# Autodesk Inventor assembly: BV-ASM-222-100 copy
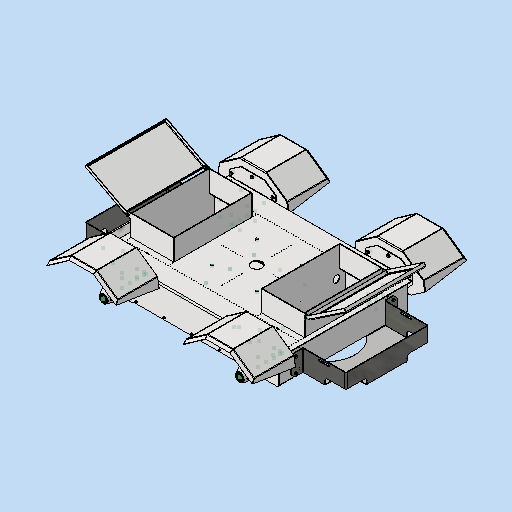
[picture p0: Inventor's stored thumbnail of the model, 512x512]
Saved by Autodesk Inventor 2025.3 (Build 293356030, 356C)
## iProperties
Created: 2025-12-05
Part Number: BV-ASM-222-100 copy
Document SubType Name: Assembly
Designer: josh
Mass: 150717 g
Surface Area: 81479.7 cm^2
Volume: 19199.6 cm^3
Density: 7.85 g/cm^3
Description: BASE VEHICLE COMPLETE ASSEMBLY
Author: josh
## iProperties of the stored document MemberDocs/x54frrunuJ0si20qmEdadrqylTg
Created: 2025-12-05
Part Number: BV-ASM-222-100 wip
Document SubType Name: Assembly
Designer: josh
Mass: 150717 g
Surface Area: 81479.7 cm^2
Volume: 19199.6 cm^3
Density: 7.85 g/cm^3
Description: BASE VEHICLE COMPLETE ASSEMBLY
Author: josh
## iProperties of the stored document MemberDocs/xFojfi5agHc25u2sk4sonpsnbLc
Created: 2025-12-05
Part Number: BV-ASM-222-100 wip
Document SubType Name: Assembly
Designer: josh
Mass: 150717 g
Surface Area: 81479.7 cm^2
Volume: 19199.6 cm^3
Density: 7.85 g/cm^3
Description: BASE VEHICLE COMPLETE ASSEMBLY
Author: josh
## Documents named in this file (59)
- R:\A1- Neuweg Design Data\OM Robotics\BASE VEHICLE DESIGN PROJECT\BV-ASM-222-100 copy.iam
- R:\A1- Neuweg Design Data\OM Robotics\BASE VEHICLE DESIGN PROJECT\BV-222-105.ipt
- R:\A1- Neuweg Design Data\OM Robotics\BASE VEHICLE DESIGN PROJECT\BV-222-106.ipt
- R:\A1- Neuweg Design Data\OM Robotics\BASE VEHICLE DESIGN PROJECT\BV-222-107.ipt
- R:\A1- Neuweg Design Data\OM Robotics\BASE VEHICLE DESIGN PROJECT\BV-222-108.ipt
- R:\A1- Neuweg Design Data\OM Robotics\BASE VEHICLE DESIGN PROJECT\BV-222-109.ipt
- R:\A1- Neuweg Design Data\OM Robotics\BASE VEHICLE DESIGN PROJECT\BV-222-112.ipt
- R:\A1- Neuweg Design Data\OM Robotics\BASE VEHICLE DESIGN PROJECT\BV-222-116.ipt
- R:\A1- Neuweg Design Data\OM Robotics\BASE VEHICLE DESIGN PROJECT\BV-222-117.ipt
- R:\A1- Neuweg Design Data\OM Robotics\BASE VEHICLE DESIGN PROJECT\BV-222-118.ipt
- R:\A1- Neuweg Design Data\OM Robotics\BASE VEHICLE DESIGN PROJECT\BV-222-119.ipt
- R:\A1- Neuweg Design Data\OM Robotics\BASE VEHICLE DESIGN PROJECT\BV-222-120.ipt
- R:\A1- Neuweg Design Data\OM Robotics\BASE VEHICLE DESIGN PROJECT\0222-110.ipt
- R:\A1- Neuweg Design Data\OM Robotics\BASE VEHICLE DESIGN PROJECT\3_8-16 x 5_8 Flange Bolt.ipt
- R:\A1- Neuweg Design Data\OM Robotics\BASE VEHICLE DESIGN PROJECT\1_4-20 UNC x 0.625.ipt
- R:\A1- Neuweg Design Data\OM Robotics\BASE VEHICLE DESIGN PROJECT\90128A277.ipt
- R:\A1- Neuweg Design Data\OM Robotics\BASE VEHICLE DESIGN PROJECT\91290A446.ipt
- R:\A1- Neuweg Design Data\OM Robotics\BASE VEHICLE DESIGN PROJECT\91259A177.ipt
- R:\A1- Neuweg Design Data\OM Robotics\BASE VEHICLE DESIGN PROJECT\94945A213.ipt
- R:\A1- Neuweg Design Data\OM Robotics\BASE VEHICLE DESIGN PROJECT\BV-ASM-222-102.iam
- R:\A1- Neuweg Design Data\OM Robotics\BASE VEHICLE DESIGN PROJECT\30205.ipt
- R:\A1- Neuweg Design Data\OM Robotics\BASE VEHICLE DESIGN PROJECT\251105 Motor_Drive.ipt
- R:\A1- Neuweg Design Data\OM Robotics\BASE VEHICLE DESIGN PROJECT\22x10x8.ipt
- R:\A1- Neuweg Design Data\OM Robotics\BASE VEHICLE DESIGN PROJECT\0222-113-2.ipt
- R:\A1- Neuweg Design Data\OM Robotics\BASE VEHICLE DESIGN PROJECT\97260A109.ipt
- R:\A1- Neuweg Design Data\OM Robotics\BASE VEHICLE DESIGN PROJECT\93560A112.ipt
- R:\A1- Neuweg Design Data\OM Robotics\BASE VEHICLE DESIGN PROJECT\1199N323.ipt
- R:\A1- Neuweg Design Data\OM Robotics\BASE VEHICLE DESIGN PROJECT\BV-ASM-222-103.iam
- R:\A1- Neuweg Design Data\OM Robotics\BASE VEHICLE DESIGN PROJECT\BV-ASM-222-104.iam
- R:\A1- Neuweg Design Data\OM Robotics\BASE VEHICLE DESIGN PROJECT\BV-ASM-222-105.iam
- C:\WORK\INVENTOR PROJECTS\misc custom projects\O&M ROBOTICS\ROBOT BASE VEHICLE\BV-222-105.ipt
- C:\WORK\INVENTOR PROJECTS\misc custom projects\O&M ROBOTICS\ROBOT BASE VEHICLE\BV-222-106.ipt
- C:\WORK\INVENTOR PROJECTS\misc custom projects\O&M ROBOTICS\ROBOT BASE VEHICLE\BV-222-107.ipt
- C:\WORK\INVENTOR PROJECTS\misc custom projects\O&M ROBOTICS\ROBOT BASE VEHICLE\BV-222-108.ipt
- C:\WORK\INVENTOR PROJECTS\misc custom projects\O&M ROBOTICS\ROBOT BASE VEHICLE\BV-222-109.ipt
- C:\WORK\INVENTOR PROJECTS\misc custom projects\O&M ROBOTICS\ROBOT BASE VEHICLE\BV-222-112.ipt
- C:\WORK\INVENTOR PROJECTS\misc custom projects\O&M ROBOTICS\ROBOT BASE VEHICLE\BV-222-116.ipt
- C:\WORK\INVENTOR PROJECTS\misc custom projects\O&M ROBOTICS\ROBOT BASE VEHICLE\BV-222-117.ipt
- C:\WORK\INVENTOR PROJECTS\misc custom projects\O&M ROBOTICS\ROBOT BASE VEHICLE\BV-222-118.ipt
- C:\WORK\INVENTOR PROJECTS\misc custom projects\O&M ROBOTICS\ROBOT BASE VEHICLE\BV-222-119.ipt
- C:\WORK\INVENTOR PROJECTS\misc custom projects\O&M ROBOTICS\ROBOT BASE VEHICLE\BV-222-120.ipt
- C:\WORK\INVENTOR PROJECTS\misc custom projects\O&M ROBOTICS\ROBOT BASE VEHICLE\0222-110.ipt
- C:\WORK\INVENTOR PROJECTS\misc custom projects\O&M ROBOTICS\ROBOT BASE VEHICLE\3_8-16 x 5_8 Flange Bolt.ipt
- C:\WORK\INVENTOR PROJECTS\misc custom projects\O&M ROBOTICS\ROBOT BASE VEHICLE\1_4-20 UNC x 0.625.ipt
- C:\WORK\INVENTOR PROJECTS\misc custom projects\O&M ROBOTICS\ROBOT BASE VEHICLE\90128A277\90128A277\90128A277.ipt
- C:\WORK\INVENTOR PROJECTS\misc custom projects\O&M ROBOTICS\ROBOT BASE VEHICLE\91290A446\91290A446\91290A446.ipt
- C:\WORK\INVENTOR PROJECTS\misc custom projects\O&M ROBOTICS\ROBOT BASE VEHICLE\91259A177\91259A177\91259A177.ipt
- C:\WORK\INVENTOR PROJECTS\misc custom projects\O&M ROBOTICS\ROBOT BASE VEHICLE\94945A213\94945A213\94945A213.ipt
- C:\WORK\INVENTOR PROJECTS\misc custom projects\O&M ROBOTICS\ROBOT BASE VEHICLE\BV-ASM-222-102.iam
- C:\WORK\INVENTOR PROJECTS\misc custom projects\O&M ROBOTICS\ROBOT BASE VEHICLE\30205\30205\30205.ipt
- C:\WORK\INVENTOR PROJECTS\misc custom projects\O&M ROBOTICS\ROBOT BASE VEHICLE\251105 Motor_Drive.ipt
- C:\WORK\INVENTOR PROJECTS\misc custom projects\O&M ROBOTICS\ROBOT BASE VEHICLE\22x10x8.ipt
- C:\WORK\INVENTOR PROJECTS\misc custom projects\O&M ROBOTICS\ROBOT BASE VEHICLE\0222-113-2.ipt
- C:\WORK\INVENTOR PROJECTS\misc custom projects\O&M ROBOTICS\ROBOT BASE VEHICLE\97260A109.ipt
- C:\WORK\INVENTOR PROJECTS\misc custom projects\O&M ROBOTICS\ROBOT BASE VEHICLE\93560A112_Steel Hex Weld Nut\93560A112_Steel Hex Weld Nut\93560A112.ipt
- C:\WORK\INVENTOR PROJECTS\misc custom projects\O&M ROBOTICS\ROBOT BASE VEHICLE\1199N323\1199N323\1199N323.ipt
- C:\WORK\INVENTOR PROJECTS\misc custom projects\O&M ROBOTICS\ROBOT BASE VEHICLE\BV-ASM-222-103.iam
- C:\WORK\INVENTOR PROJECTS\misc custom projects\O&M ROBOTICS\ROBOT BASE VEHICLE\BV-ASM-222-104.iam
- C:\WORK\INVENTOR PROJECTS\misc custom projects\O&M ROBOTICS\ROBOT BASE VEHICLE\BV-ASM-222-105.iam
## Components (199 placed, 29 different names)
1. BV-ASM-222-104:1 [sub-assembly] — Flush:11, Flush:12, Flush:13
2. BV-ASM-222-105:1 [sub-assembly] — Mate:105
3. BV-ASM-222-103:1 [sub-assembly] — Flush:8, Flush:9, Flush:10, Insert:201, Insert:202
4. BV-ASM-222-103:2 [sub-assembly] — Insert:203, Insert:204, Insert:205, Insert:206, Insert:219, Insert:220
5. BV-ASM-222-103:3 [sub-assembly] — Insert:207, Insert:208, Insert:209, Insert:210, Insert:221, Insert:222
6. BV-ASM-222-103:4 [sub-assembly] — Insert:211, Insert:212, Insert:213, Insert:214, Insert:223, Insert:224
7. BV-222-105:1 — Insert:117, Insert:118, Insert:119, Insert:120, Insert:121, Insert:122, Insert:123, Insert:124, Insert:125, Insert:126, Insert:127, Insert:128
8. BV-222-106:1 — Mate:2, Insert:162, Insert:166
9. BV-222-107:1 — Insert:161, Insert:165
10. BV-222-108:1 — Mate:2, Flush:1, Mate:3
11. BV-222-109:1 — Insert:75, Insert:76, Insert:77, Insert:201, Insert:202
12. BV-222-112:1 — Mate:73, Mate:74, Mate:75, Mate:76, Mate:77, Mate:78, Mate:79, Mate:80, Mate:81, Mate:82, Mate:83, Mate:84, Mate:85, Mate:86, Mate:87, Mate:88, Mate:89, Mate:90, Mate:91, Mate:92
13. BV-222-116:1 — Insert:174, Insert:189
14. BV-222-118:1
15. BV-222-119:1 — Insert:175, Insert:190
16. BV-222-120:1 — Mate:5
17. BV-222-112:3
18. BV-222-106:2 — Mate:1, Insert:163, Insert:168
19. BV-222-107:2 — Insert:164, Insert:167
20. BV-222-108:2 — Mate:1, Mate:3
21. BV-222-109:2 — Insert:78, Insert:79, Insert:80, Insert:203, Insert:204, Insert:219, Insert:220
22. BV-222-116:2 — Insert:173, Insert:185
23. BV-222-118:2
24. BV-222-119:2 — Insert:176, Insert:186
25. BV-222-120:2
26. BV-222-109:3 — Insert:81, Insert:82, Insert:83, Insert:211, Insert:212, Insert:223, Insert:224
27. BV-222-116:3 — Insert:170, Insert:192
28. BV-222-118:3
29. BV-222-119:3 — Insert:169, Insert:191
30. BV-222-120:3 — Mate:14
31. BV-222-109:4 — Insert:84, Insert:85, Insert:86, Insert:207, Insert:208, Insert:221, Insert:222
32. BV-222-116:4 — Insert:172, Insert:188
33. BV-222-118:4
34. BV-222-119:4 — Insert:171, Insert:187
35. BV-222-120:4 — Mate:11
36. BV-ASM-222-102:1 [sub-assembly] — Mate:12, Mate:13, Insert:30, Insert:31, Insert:215
37. BV-ASM-222-102:2 [sub-assembly] — Mate:4, Mate:6, Insert:16, Insert:17, Mate:102, Insert:217
38. BV-ASM-222-102:3 [sub-assembly] — Mate:9, Mate:10, Insert:28, Insert:29, Mate:103, Insert:218
39. BV-ASM-222-102:4 [sub-assembly] — Mate:7, Mate:8, Insert:22, Insert:23, Mate:101, Insert:216
40. 251105 Motor_Drive:1 — Mate:4, Mate:5, Mate:6, Flush:2, Flush:3, Mate:102
41. 22x10x8:1 — Insert:16, Insert:17
42. 97260A109:1 — Insert:196
43. 251105 Motor_Drive:2 — Mate:7, Flush:2, Flush:3, Mate:8, Flush:4, Mate:101
44. 97260A109:2 — Insert:194
45. 22x10x8:2 — Insert:22, Insert:23
46. 251105 Motor_Drive:3 — Mate:9, Mate:10, Mate:11, Flush:4, Flush:5, Mate:103
47. 251105 Motor_Drive:4 — Mate:12, Mate:13, Mate:14, Flush:5
48. 97260A109:3 — Insert:200
49. 97260A109:4 — Insert:198
50. 22x10x8:3 — Insert:28, Insert:29
51. 22x10x8:4 — Insert:30, Insert:31
52. 93560A112:1
53. 93560A112:2
54. 93560A112:3
55. 93560A112:4
56. 0222-110:1 — Mate:104, Flush:7
57. 0222-110:2 — Flush:7, Flush:19, Mate:105
58. Hex Flange Screw - Inch (IFI) 3/8-16 UNC x 0.625:9
59. Hex Flange Screw - Inch (IFI) 3/8-16 UNC x 0.625:10
60. Hex Flange Screw - Inch (IFI) 3/8-16 UNC x 0.625:11
61. Hex Flange Screw - Inch (IFI) 3/8-16 UNC x 0.625:12
62. Hex Flange Screw - Inch (IFI) 3/8-16 UNC x 0.625:13
63. Hex Flange Screw - Inch (IFI) 3/8-16 UNC x 0.625:14
64. Hex Flange Screw - Inch (IFI) 3/8-16 UNC x 0.625:15
65. Hex Flange Screw - Inch (IFI) 3/8-16 UNC x 0.625:16
66. Hex Flange Screw - Inch (IFI) 3/8-16 UNC x 0.625:18 — Insert:75, Mate:21, Mate:22
67. Hex Flange Screw - Inch (IFI) 3/8-16 UNC x 0.625:19 — Insert:76, Mate:21, Mate:22
68. Hex Flange Screw - Inch (IFI) 3/8-16 UNC x 0.625:20 — Insert:77, Mate:23, Mate:24
69. Hex Flange Screw - Inch (IFI) 3/8-16 UNC x 0.625:21 — Insert:78, Mate:23, Mate:24
70. Hex Flange Screw - Inch (IFI) 3/8-16 UNC x 0.625:22 — Insert:79, Mate:25, Mate:26
71. Hex Flange Screw - Inch (IFI) 3/8-16 UNC x 0.625:23 — Insert:80, Mate:25, Mate:26
72. Hex Flange Screw - Inch (IFI) 3/8-16 UNC x 0.625:24 — Insert:81, Mate:27, Mate:28
73. Hex Flange Screw - Inch (IFI) 3/8-16 UNC x 0.625:25 — Insert:82, Mate:27, Mate:28
74. Hex Flange Screw - Inch (IFI) 3/8-16 UNC x 0.625:26 — Insert:83, Mate:29, Mate:30
75. Hex Flange Screw - Inch (IFI) 3/8-16 UNC x 0.625:27 — Insert:84, Mate:29, Mate:30
76. Hex Flange Screw - Inch (IFI) 3/8-16 UNC x 0.625:28 — Insert:85, Mate:31, Mate:32
77. Hex Flange Screw - Inch (IFI) 3/8-16 UNC x 0.625:29 — Insert:86, Mate:31, Mate:32
78. Hex Flange Screw - Inch (IFI) 3/8-16 UNC x 0.625:30 — Mate:33, Mate:34
79. Hex Flange Screw - Inch (IFI) 3/8-16 UNC x 0.625:31 — Mate:33, Mate:34
80. Hex Flange Screw - Inch (IFI) 3/8-16 UNC x 0.625:32 — Mate:35, Mate:36, Insert:205
81. Hex Flange Screw - Inch (IFI) 3/8-16 UNC x 0.625:33 — Mate:35, Mate:36, Insert:206
82. Hex Flange Screw - Inch (IFI) 3/8-16 UNC x 0.625:34 — Mate:37, Mate:38, Insert:214
83. Hex Flange Screw - Inch (IFI) 3/8-16 UNC x 0.625:35 — Mate:37, Mate:38, Insert:213
84. Hex Flange Screw - Inch (IFI) 3/8-16 UNC x 0.625:36 — Mate:39, Mate:40, Insert:209
85. Hex Flange Screw - Inch (IFI) 3/8-16 UNC x 0.625:37 — Mate:39, Mate:40, Insert:210
86. 1_4-20 UNC x 0.625:1 — Mate:41, Mate:42
87. 1_4-20 UNC x 0.625:2 — Mate:41, Mate:42
88. 1_4-20 UNC x 0.625:3 — Mate:43, Mate:44
89. 1_4-20 UNC x 0.625:4 — Mate:43, Mate:44
90. 1_4-20 UNC x 0.625:5 — Mate:45, Mate:46
91. 1_4-20 UNC x 0.625:6 — Mate:45, Mate:46
92. 1_4-20 UNC x 0.625:7 — Mate:47, Mate:48
93. 1_4-20 UNC x 0.625:8 — Mate:47, Mate:48
94. 1_4-20 UNC x 0.625:9 — Mate:49, Mate:50
95. 1_4-20 UNC x 0.625:10 — Mate:49, Mate:50
96. Hex Flange Screw - Inch (IFI) 3/8-16 UNC x 0.625:38 — Insert:117, Mate:51, Mate:52
97. Hex Flange Screw - Inch (IFI) 3/8-16 UNC x 0.625:39 — Insert:118, Mate:51, Mate:52
98. Hex Flange Screw - Inch (IFI) 3/8-16 UNC x 0.625:40 — Insert:119, Mate:53, Mate:54
99. Hex Flange Screw - Inch (IFI) 3/8-16 UNC x 0.625:41 — Insert:120, Mate:53, Mate:54
100. Hex Flange Screw - Inch (IFI) 3/8-16 UNC x 0.625:42 — Insert:121, Mate:55, Mate:56
101. Hex Flange Screw - Inch (IFI) 3/8-16 UNC x 0.625:43 — Insert:122, Mate:55, Mate:56
102. Hex Flange Screw - Inch (IFI) 3/8-16 UNC x 0.625:44 — Insert:123, Mate:57, Mate:58
103. Hex Flange Screw - Inch (IFI) 3/8-16 UNC x 0.625:45 — Insert:124, Mate:57, Mate:58
104. Hex Flange Screw - Inch (IFI) 3/8-16 UNC x 0.625:46 — Insert:125, Mate:59, Mate:60
105. Hex Flange Screw - Inch (IFI) 3/8-16 UNC x 0.625:47 — Insert:126, Mate:59, Mate:60
106. Hex Flange Screw - Inch (IFI) 3/8-16 UNC x 0.625:48 — Insert:127, Mate:61, Mate:62
107. Hex Flange Screw - Inch (IFI) 3/8-16 UNC x 0.625:49 — Insert:128, Mate:61, Mate:62
108. 1_4-20 UNC x 0.625:11 — Mate:75, Mate:76
109. 1_4-20 UNC x 0.625:12 — Mate:89, Mate:90
110. 1_4-20 UNC x 0.625:13 — Mate:77, Mate:78
111. 1_4-20 UNC x 0.625:14 — Mate:81, Mate:82
112. 1_4-20 UNC x 0.625:15 — Mate:79, Mate:80
113. 1_4-20 UNC x 0.625:16 — Mate:91, Mate:92
114. 1_4-20 UNC x 0.625:17 — Mate:85, Mate:86
115. 1_4-20 UNC x 0.625:18 — Mate:83, Mate:84
116. 1_4-20 UNC x 0.625:19 — Mate:87, Mate:88
117. 1_4-20 UNC x 0.625:20 — Mate:73, Mate:74
118. 1_4-20 UNC x 0.625:21 — Mate:93, Mate:94
119. 1_4-20 UNC x 0.625:22 — Mate:93, Mate:94
120. 1_4-20 UNC x 0.625:23 — Mate:95, Mate:96
121. 1_4-20 UNC x 0.625:24 — Mate:95, Mate:96
122. 1_4-20 UNC x 0.625:25
123. 1_4-20 UNC x 0.625:26
124. 1_4-20 UNC x 0.625:27 — Mate:97, Mate:98
125. 1_4-20 UNC x 0.625:28 — Mate:97, Mate:98
126. 1_4-20 UNC x 0.625:29 — Mate:99, Mate:100
127. 1_4-20 UNC x 0.625:30 — Mate:99, Mate:100
128. 90128A277:1
129. 90128A277:2
130. 90128A277:3
131. 90128A277:4
132. 90128A277:5
133. 90128A277:6
134. 90128A277:7
135. 90128A277:8
136. 90128A277:9
137. 90128A277:10
138. 90128A277:11
139. 90128A277:12
140. 90128A277:13
141. 90128A277:14
142. 90128A277:15
143. 90128A277:16
144. 91290A446:1
145. 91290A446:2
146. 91290A446:3
147. 91290A446:4
148. 91290A446:5
149. 91290A446:6
150. 91290A446:7
151. 91290A446:8
152. 91290A446:9
153. 91290A446:10
154. 91290A446:11
155. 91290A446:12
156. 91290A446:13
157. 91290A446:14
158. 91290A446:15
159. 91290A446:16
160. 91259A177:1 — Insert:162
161. 91259A177:2 — Insert:161
162. 91259A177:3 — Insert:163
163. 91259A177:4 — Insert:164
164. 94945A213:1 — Insert:165
165. 94945A213:2 — Insert:166
166. 94945A213:3 — Insert:167
167. 94945A213:4 — Insert:168
168. 30205:1 — Insert:170, Insert:215
169. 30205:2 — Insert:169, Insert:197
170. 30205:3 — Insert:172, Insert:218
171. 30205:4 — Insert:171, Insert:199
172. 30205:5 — Insert:176, Insert:193
173. 30205:6 — Insert:173, Insert:216
174. 30205:7 — Insert:175, Insert:195
175. 30205:8 — Insert:174, Insert:217
176. 0222-113-2:1 — Insert:199, Insert:200
177. 0222-113-2:2 — Insert:193, Insert:194
178. 0222-113-2:3 — Insert:197, Insert:198
179. 0222-113-2:4 — Insert:195, Insert:196
180. 1199N323:1 — Insert:185
181. 1199N323:2 — Insert:186
182. 1199N323:3 — Insert:187
183. 1199N323:4 — Insert:188
184. 1199N323:5 — Insert:189
185. 1199N323:6 — Insert:190
186. 1199N323:7 — Insert:191
187. 1199N323:8 — Insert:192
188. BV-222-117:1
189. BV-222-117:2
190. BV-222-117:3
191. BV-222-117:4
192. BV-222-117:5
193. BV-222-117:6
194. BV-222-117:7
195. BV-222-117:9
196. BV-222-117:10
197. BV-222-117:8
198. BV-222-117:11
199. BV-222-117:12
## Component patterns: (3 elements, first: BV-222-117:1), (3 elements, first: BV-222-117:4), (3 elements, first: BV-222-117:7), (3 elements, first: BV-222-117:8)
## Relationships (259: Insert 146, Mate 99, Flush 13, Angle 1)
- [Insert]: BV-ASM-222-104:1 ↔ BV-222-112:3
- [Insert]: BV-ASM-222-104:1 ↔ BV-222-112:3
- Mate:1: BV-222-106:2 ↔ BV-222-108:2
- Mate:2: BV-222-106:1 ↔ BV-222-108:1
- Flush:1: BV-222-108:1
- Mate:3: BV-222-108:1 ↔ BV-222-108:2
- Mate:4: BV-ASM-222-102:2 ↔ 251105 Motor_Drive:1
- Mate:5: BV-222-120:1 ↔ 251105 Motor_Drive:1
- Mate:6: BV-ASM-222-102:2 ↔ 251105 Motor_Drive:1
- Insert:16: BV-ASM-222-102:2 ↔ 22x10x8:1
- Insert:17: BV-ASM-222-102:2 ↔ 22x10x8:1
- [Angle] (-90 deg): BV-ASM-222-105:1 ↔ 251105 Motor_Drive:1
- Mate:7: BV-ASM-222-102:4 ↔ 251105 Motor_Drive:2
- Flush:2: 251105 Motor_Drive:1 ↔ 251105 Motor_Drive:2
- Flush:3: 251105 Motor_Drive:1 ↔ 251105 Motor_Drive:2
- Mate:8: BV-ASM-222-102:4 ↔ 251105 Motor_Drive:2
- Insert:22: BV-ASM-222-102:4 ↔ 22x10x8:2
- Insert:23: BV-ASM-222-102:4 ↔ 22x10x8:2
- Mate:9: BV-ASM-222-102:3 ↔ 251105 Motor_Drive:3
- Mate:10: BV-ASM-222-102:3 ↔ 251105 Motor_Drive:3
- Mate:11: BV-222-120:4 ↔ 251105 Motor_Drive:3
- Flush:4: 251105 Motor_Drive:2 ↔ 251105 Motor_Drive:3
- Mate:12: BV-ASM-222-102:1 ↔ 251105 Motor_Drive:4
- Mate:13: BV-ASM-222-102:1 ↔ 251105 Motor_Drive:4
- Mate:14: BV-222-120:3 ↔ 251105 Motor_Drive:4
- Flush:5: 251105 Motor_Drive:3 ↔ 251105 Motor_Drive:4
- Insert:28: BV-ASM-222-102:3 ↔ 22x10x8:3
- Insert:29: BV-ASM-222-102:3 ↔ 22x10x8:3
- Insert:30: BV-ASM-222-102:1 ↔ 22x10x8:4
- Insert:31: BV-ASM-222-102:1 ↔ 22x10x8:4
- [Insert]: BV-ASM-222-105:1 ↔ 93560A112:1
- [Insert]: BV-ASM-222-105:1 ↔ 93560A112:2
- [Insert]: BV-ASM-222-105:1 ↔ 93560A112:3
- [Insert]: BV-ASM-222-105:1 ↔ 93560A112:4
- [Mate]: BV-ASM-222-105:1 ↔ 0222-110:1
- Mate:104: 0222-110:1
- [Mate]: BV-ASM-222-105:1 ↔ 0222-110:1
- Flush:7: 0222-110:1 ↔ 0222-110:2
- Flush:19: 0222-110:2
- [Insert] (4.7752 mm): BV-ASM-222-105:1 ↔ Hex Flange Screw - Inch (IFI) 3/8-16 UNC x 0.625:9
- [Insert] (4.7752 mm): BV-ASM-222-105:1 ↔ Hex Flange Screw - Inch (IFI) 3/8-16 UNC x 0.625:10
- [Insert] (4.7752 mm): BV-ASM-222-105:1 ↔ Hex Flange Screw - Inch (IFI) 3/8-16 UNC x 0.625:12
- [Insert] (4.7752 mm): BV-ASM-222-105:1 ↔ Hex Flange Screw - Inch (IFI) 3/8-16 UNC x 0.625:11
- [Insert] (4.7752 mm): BV-ASM-222-105:1 ↔ Hex Flange Screw - Inch (IFI) 3/8-16 UNC x 0.625:16
- [Insert] (4.7752 mm): BV-ASM-222-105:1 ↔ Hex Flange Screw - Inch (IFI) 3/8-16 UNC x 0.625:15
- [Insert] (4.7752 mm): BV-ASM-222-105:1 ↔ Hex Flange Screw - Inch (IFI) 3/8-16 UNC x 0.625:14
- [Insert] (4.7752 mm): BV-ASM-222-105:1 ↔ Hex Flange Screw - Inch (IFI) 3/8-16 UNC x 0.625:13
- Insert:75: BV-222-109:1 ↔ Hex Flange Screw - Inch (IFI) 3/8-16 UNC x 0.625:18
- Insert:76: BV-222-109:1 ↔ Hex Flange Screw - Inch (IFI) 3/8-16 UNC x 0.625:19
- Mate:21: Hex Flange Screw - Inch (IFI) 3/8-16 UNC x 0.625:18 ↔ Hex Flange Screw - Inch (IFI) 3/8-16 UNC x 0.625:19
- Mate:22: Hex Flange Screw - Inch (IFI) 3/8-16 UNC x 0.625:18 ↔ Hex Flange Screw - Inch (IFI) 3/8-16 UNC x 0.625:19
- Insert:77: BV-222-109:1 ↔ Hex Flange Screw - Inch (IFI) 3/8-16 UNC x 0.625:20
- Insert:78: BV-222-109:2 ↔ Hex Flange Screw - Inch (IFI) 3/8-16 UNC x 0.625:21
- Mate:23: Hex Flange Screw - Inch (IFI) 3/8-16 UNC x 0.625:20 ↔ Hex Flange Screw - Inch (IFI) 3/8-16 UNC x 0.625:21
- Mate:24: Hex Flange Screw - Inch (IFI) 3/8-16 UNC x 0.625:20 ↔ Hex Flange Screw - Inch (IFI) 3/8-16 UNC x 0.625:21
- Insert:79: BV-222-109:2 ↔ Hex Flange Screw - Inch (IFI) 3/8-16 UNC x 0.625:22
- Insert:80: BV-222-109:2 ↔ Hex Flange Screw - Inch (IFI) 3/8-16 UNC x 0.625:23
- Mate:25: Hex Flange Screw - Inch (IFI) 3/8-16 UNC x 0.625:22 ↔ Hex Flange Screw - Inch (IFI) 3/8-16 UNC x 0.625:23
- Mate:26: Hex Flange Screw - Inch (IFI) 3/8-16 UNC x 0.625:22 ↔ Hex Flange Screw - Inch (IFI) 3/8-16 UNC x 0.625:23
- Insert:81: BV-222-109:3 ↔ Hex Flange Screw - Inch (IFI) 3/8-16 UNC x 0.625:24
- Insert:82: BV-222-109:3 ↔ Hex Flange Screw - Inch (IFI) 3/8-16 UNC x 0.625:25
- Mate:27: Hex Flange Screw - Inch (IFI) 3/8-16 UNC x 0.625:24 ↔ Hex Flange Screw - Inch (IFI) 3/8-16 UNC x 0.625:25
- Mate:28: Hex Flange Screw - Inch (IFI) 3/8-16 UNC x 0.625:24 ↔ Hex Flange Screw - Inch (IFI) 3/8-16 UNC x 0.625:25
- Insert:83: BV-222-109:3 ↔ Hex Flange Screw - Inch (IFI) 3/8-16 UNC x 0.625:26
- Insert:84: BV-222-109:4 ↔ Hex Flange Screw - Inch (IFI) 3/8-16 UNC x 0.625:27
- Mate:29: Hex Flange Screw - Inch (IFI) 3/8-16 UNC x 0.625:26 ↔ Hex Flange Screw - Inch (IFI) 3/8-16 UNC x 0.625:27
- Mate:30: Hex Flange Screw - Inch (IFI) 3/8-16 UNC x 0.625:26 ↔ Hex Flange Screw - Inch (IFI) 3/8-16 UNC x 0.625:27
- Insert:85: BV-222-109:4 ↔ Hex Flange Screw - Inch (IFI) 3/8-16 UNC x 0.625:28
- Insert:86: BV-222-109:4 ↔ Hex Flange Screw - Inch (IFI) 3/8-16 UNC x 0.625:29
- Mate:31: Hex Flange Screw - Inch (IFI) 3/8-16 UNC x 0.625:28 ↔ Hex Flange Screw - Inch (IFI) 3/8-16 UNC x 0.625:29
- Mate:32: Hex Flange Screw - Inch (IFI) 3/8-16 UNC x 0.625:28 ↔ Hex Flange Screw - Inch (IFI) 3/8-16 UNC x 0.625:29
- [Insert]: BV-ASM-222-103:1 ↔ Hex Flange Screw - Inch (IFI) 3/8-16 UNC x 0.625:30
- [Insert]: BV-ASM-222-103:1 ↔ Hex Flange Screw - Inch (IFI) 3/8-16 UNC x 0.625:31
- Mate:33: Hex Flange Screw - Inch (IFI) 3/8-16 UNC x 0.625:30 ↔ Hex Flange Screw - Inch (IFI) 3/8-16 UNC x 0.625:31
- Mate:34: Hex Flange Screw - Inch (IFI) 3/8-16 UNC x 0.625:30 ↔ Hex Flange Screw - Inch (IFI) 3/8-16 UNC x 0.625:31
- Mate:35: Hex Flange Screw - Inch (IFI) 3/8-16 UNC x 0.625:32 ↔ Hex Flange Screw - Inch (IFI) 3/8-16 UNC x 0.625:33
- Mate:36: Hex Flange Screw - Inch (IFI) 3/8-16 UNC x 0.625:32 ↔ Hex Flange Screw - Inch (IFI) 3/8-16 UNC x 0.625:33
- Mate:37: Hex Flange Screw - Inch (IFI) 3/8-16 UNC x 0.625:34 ↔ Hex Flange Screw - Inch (IFI) 3/8-16 UNC x 0.625:35
- Mate:38: Hex Flange Screw - Inch (IFI) 3/8-16 UNC x 0.625:34 ↔ Hex Flange Screw - Inch (IFI) 3/8-16 UNC x 0.625:35
- Mate:39: Hex Flange Screw - Inch (IFI) 3/8-16 UNC x 0.625:36 ↔ Hex Flange Screw - Inch (IFI) 3/8-16 UNC x 0.625:37
- Mate:40: Hex Flange Screw - Inch (IFI) 3/8-16 UNC x 0.625:36 ↔ Hex Flange Screw - Inch (IFI) 3/8-16 UNC x 0.625:37
- [Insert]: BV-ASM-222-104:1 ↔ 1_4-20 UNC x 0.625:1
- [Insert]: BV-ASM-222-104:1 ↔ 1_4-20 UNC x 0.625:2
- Mate:41: 1_4-20 UNC x 0.625:1 ↔ 1_4-20 UNC x 0.625:2
- Mate:42: 1_4-20 UNC x 0.625:1 ↔ 1_4-20 UNC x 0.625:2
- [Insert]: BV-ASM-222-104:1 ↔ 1_4-20 UNC x 0.625:3
- [Insert]: BV-ASM-222-104:1 ↔ 1_4-20 UNC x 0.625:4
- Mate:43: 1_4-20 UNC x 0.625:3 ↔ 1_4-20 UNC x 0.625:4
- Mate:44: 1_4-20 UNC x 0.625:3 ↔ 1_4-20 UNC x 0.625:4
- [Insert]: BV-ASM-222-104:1 ↔ 1_4-20 UNC x 0.625:5
- [Insert]: BV-ASM-222-104:1 ↔ 1_4-20 UNC x 0.625:6
- Mate:45: 1_4-20 UNC x 0.625:5 ↔ 1_4-20 UNC x 0.625:6
- Mate:46: 1_4-20 UNC x 0.625:5 ↔ 1_4-20 UNC x 0.625:6
- [Insert]: BV-ASM-222-104:1 ↔ 1_4-20 UNC x 0.625:7
- [Insert]: BV-ASM-222-104:1 ↔ 1_4-20 UNC x 0.625:8
- Mate:47: 1_4-20 UNC x 0.625:7 ↔ 1_4-20 UNC x 0.625:8
- Mate:48: 1_4-20 UNC x 0.625:7 ↔ 1_4-20 UNC x 0.625:8
- [Insert]: BV-ASM-222-104:1 ↔ 1_4-20 UNC x 0.625:9
- [Insert]: BV-ASM-222-104:1 ↔ 1_4-20 UNC x 0.625:10
- Mate:49: 1_4-20 UNC x 0.625:9 ↔ 1_4-20 UNC x 0.625:10
- Mate:50: 1_4-20 UNC x 0.625:9 ↔ 1_4-20 UNC x 0.625:10
- Insert:117: BV-222-105:1 ↔ Hex Flange Screw - Inch (IFI) 3/8-16 UNC x 0.625:38
- Insert:118: BV-222-105:1 ↔ Hex Flange Screw - Inch (IFI) 3/8-16 UNC x 0.625:39
- Mate:51: Hex Flange Screw - Inch (IFI) 3/8-16 UNC x 0.625:38 ↔ Hex Flange Screw - Inch (IFI) 3/8-16 UNC x 0.625:39
- Mate:52: Hex Flange Screw - Inch (IFI) 3/8-16 UNC x 0.625:38 ↔ Hex Flange Screw - Inch (IFI) 3/8-16 UNC x 0.625:39
- Insert:119: BV-222-105:1 ↔ Hex Flange Screw - Inch (IFI) 3/8-16 UNC x 0.625:40
- Insert:120: BV-222-105:1 ↔ Hex Flange Screw - Inch (IFI) 3/8-16 UNC x 0.625:41
- Mate:53: Hex Flange Screw - Inch (IFI) 3/8-16 UNC x 0.625:40 ↔ Hex Flange Screw - Inch (IFI) 3/8-16 UNC x 0.625:41
- Mate:54: Hex Flange Screw - Inch (IFI) 3/8-16 UNC x 0.625:40 ↔ Hex Flange Screw - Inch (IFI) 3/8-16 UNC x 0.625:41
- Insert:121: BV-222-105:1 ↔ Hex Flange Screw - Inch (IFI) 3/8-16 UNC x 0.625:42
- Insert:122: BV-222-105:1 ↔ Hex Flange Screw - Inch (IFI) 3/8-16 UNC x 0.625:43
- Mate:55: Hex Flange Screw - Inch (IFI) 3/8-16 UNC x 0.625:42 ↔ Hex Flange Screw - Inch (IFI) 3/8-16 UNC x 0.625:43
- Mate:56: Hex Flange Screw - Inch (IFI) 3/8-16 UNC x 0.625:42 ↔ Hex Flange Screw - Inch (IFI) 3/8-16 UNC x 0.625:43
- Insert:123: BV-222-105:1 ↔ Hex Flange Screw - Inch (IFI) 3/8-16 UNC x 0.625:44
- Insert:124: BV-222-105:1 ↔ Hex Flange Screw - Inch (IFI) 3/8-16 UNC x 0.625:45
- Mate:57: Hex Flange Screw - Inch (IFI) 3/8-16 UNC x 0.625:44 ↔ Hex Flange Screw - Inch (IFI) 3/8-16 UNC x 0.625:45
- Mate:58: Hex Flange Screw - Inch (IFI) 3/8-16 UNC x 0.625:44 ↔ Hex Flange Screw - Inch (IFI) 3/8-16 UNC x 0.625:45
- Insert:125: BV-222-105:1 ↔ Hex Flange Screw - Inch (IFI) 3/8-16 UNC x 0.625:46
- Insert:126: BV-222-105:1 ↔ Hex Flange Screw - Inch (IFI) 3/8-16 UNC x 0.625:47
- Mate:59: Hex Flange Screw - Inch (IFI) 3/8-16 UNC x 0.625:46 ↔ Hex Flange Screw - Inch (IFI) 3/8-16 UNC x 0.625:47
- Mate:60: Hex Flange Screw - Inch (IFI) 3/8-16 UNC x 0.625:46 ↔ Hex Flange Screw - Inch (IFI) 3/8-16 UNC x 0.625:47
- Insert:127: BV-222-105:1 ↔ Hex Flange Screw - Inch (IFI) 3/8-16 UNC x 0.625:48
- Insert:128: BV-222-105:1 ↔ Hex Flange Screw - Inch (IFI) 3/8-16 UNC x 0.625:49
- Mate:61: Hex Flange Screw - Inch (IFI) 3/8-16 UNC x 0.625:48 ↔ Hex Flange Screw - Inch (IFI) 3/8-16 UNC x 0.625:49
- Mate:62: Hex Flange Screw - Inch (IFI) 3/8-16 UNC x 0.625:48 ↔ Hex Flange Screw - Inch (IFI) 3/8-16 UNC x 0.625:49
- [Mate]: 1_4-20 UNC x 0.625:11 ↔ 1_4-20 UNC x 0.625:12
- [Mate]: 1_4-20 UNC x 0.625:11 ↔ 1_4-20 UNC x 0.625:12
- [Mate]: 1_4-20 UNC x 0.625:13 ↔ 1_4-20 UNC x 0.625:14
- [Mate]: 1_4-20 UNC x 0.625:13 ↔ 1_4-20 UNC x 0.625:14
- [Mate]: 1_4-20 UNC x 0.625:17 ↔ 1_4-20 UNC x 0.625:18
- [Mate]: 1_4-20 UNC x 0.625:17 ↔ 1_4-20 UNC x 0.625:18
- [Mate]: 1_4-20 UNC x 0.625:19 ↔ 1_4-20 UNC x 0.625:20
- [Mate]: 1_4-20 UNC x 0.625:19 ↔ 1_4-20 UNC x 0.625:20
- Mate:73: BV-222-112:1 ↔ 1_4-20 UNC x 0.625:20
- Mate:74: BV-222-112:1 ↔ 1_4-20 UNC x 0.625:20
- Mate:75: BV-222-112:1 ↔ 1_4-20 UNC x 0.625:11
- Mate:76: BV-222-112:1 ↔ 1_4-20 UNC x 0.625:11
- Mate:77: BV-222-112:1 ↔ 1_4-20 UNC x 0.625:13
- Mate:78: BV-222-112:1 ↔ 1_4-20 UNC x 0.625:13
- Mate:79: BV-222-112:1 ↔ 1_4-20 UNC x 0.625:15
- Mate:80: BV-222-112:1 ↔ 1_4-20 UNC x 0.625:15
- Mate:81: BV-222-112:1 ↔ 1_4-20 UNC x 0.625:14
- Mate:82: BV-222-112:1 ↔ 1_4-20 UNC x 0.625:14
- Mate:83: BV-222-112:1 ↔ 1_4-20 UNC x 0.625:18
- Mate:84: BV-222-112:1 ↔ 1_4-20 UNC x 0.625:18
- Mate:85: BV-222-112:1 ↔ 1_4-20 UNC x 0.625:17
- Mate:86: BV-222-112:1 ↔ 1_4-20 UNC x 0.625:17
- Mate:87: BV-222-112:1 ↔ 1_4-20 UNC x 0.625:19
- Mate:88: BV-222-112:1 ↔ 1_4-20 UNC x 0.625:19
- Mate:89: BV-222-112:1 ↔ 1_4-20 UNC x 0.625:12
- Mate:90: BV-222-112:1 ↔ 1_4-20 UNC x 0.625:12
- Mate:91: BV-222-112:1 ↔ 1_4-20 UNC x 0.625:16
- Mate:92: BV-222-112:1 ↔ 1_4-20 UNC x 0.625:16
- Mate:93: 1_4-20 UNC x 0.625:21 ↔ 1_4-20 UNC x 0.625:22
- Mate:94: 1_4-20 UNC x 0.625:21 ↔ 1_4-20 UNC x 0.625:22
- Mate:95: 1_4-20 UNC x 0.625:23 ↔ 1_4-20 UNC x 0.625:24
- Mate:96: 1_4-20 UNC x 0.625:23 ↔ 1_4-20 UNC x 0.625:24
- Mate:97: 1_4-20 UNC x 0.625:27 ↔ 1_4-20 UNC x 0.625:28
- Mate:98: 1_4-20 UNC x 0.625:27 ↔ 1_4-20 UNC x 0.625:28
- Mate:99: 1_4-20 UNC x 0.625:29 ↔ 1_4-20 UNC x 0.625:30
- Mate:100: 1_4-20 UNC x 0.625:29 ↔ 1_4-20 UNC x 0.625:30
- [Insert]: BV-ASM-222-104:1 ↔ 90128A277:1
- [Insert]: BV-ASM-222-104:1 ↔ 90128A277:2
- [Insert]: BV-ASM-222-104:1 ↔ 90128A277:3
- [Insert]: BV-ASM-222-104:1 ↔ 90128A277:4
- [Insert]: BV-ASM-222-104:1 ↔ 90128A277:5
- [Insert]: BV-ASM-222-104:1 ↔ 90128A277:6
- [Insert]: BV-ASM-222-104:1 ↔ 90128A277:7
- [Insert]: BV-ASM-222-104:1 ↔ 90128A277:8
- [Insert]: BV-ASM-222-104:1 ↔ 90128A277:9
- [Insert]: BV-ASM-222-104:1 ↔ 90128A277:10
- [Insert]: BV-ASM-222-104:1 ↔ 90128A277:11
- [Insert]: BV-ASM-222-104:1 ↔ 90128A277:12
- [Insert]: BV-ASM-222-104:1 ↔ 90128A277:13
- [Insert]: BV-ASM-222-104:1 ↔ 90128A277:14
- [Insert]: BV-ASM-222-104:1 ↔ 90128A277:15
- [Insert]: BV-ASM-222-104:1 ↔ 90128A277:16
- [Insert]: BV-ASM-222-105:1 ↔ 91290A446:1
- [Insert]: BV-ASM-222-105:1 ↔ 91290A446:2
- [Insert]: BV-ASM-222-105:1 ↔ 91290A446:3
- [Insert]: BV-ASM-222-105:1 ↔ 91290A446:4
- [Insert]: BV-ASM-222-105:1 ↔ 91290A446:5
- [Insert]: BV-ASM-222-105:1 ↔ 91290A446:6
- [Insert]: BV-ASM-222-105:1 ↔ 91290A446:7
- [Insert]: BV-ASM-222-105:1 ↔ 91290A446:8
- [Insert]: BV-ASM-222-105:1 ↔ 91290A446:9
- [Insert]: BV-ASM-222-105:1 ↔ 91290A446:10
- [Insert]: BV-ASM-222-105:1 ↔ 91290A446:11
- [Insert]: BV-ASM-222-105:1 ↔ 91290A446:12
- [Insert]: BV-ASM-222-105:1 ↔ 91290A446:13
- [Insert]: BV-ASM-222-105:1 ↔ 91290A446:14
- [Insert]: BV-ASM-222-105:1 ↔ 91290A446:15
- [Insert]: BV-ASM-222-105:1 ↔ 91290A446:16
- Insert:161: BV-222-107:1 ↔ 91259A177:2
- Insert:162: BV-222-106:1 ↔ 91259A177:1
- Insert:163: BV-222-106:2 ↔ 91259A177:3
- Insert:164: BV-222-107:2 ↔ 91259A177:4
- Insert:165: BV-222-107:1 ↔ 94945A213:1
- Insert:166: BV-222-106:1 ↔ 94945A213:2
- Insert:167: BV-222-107:2 ↔ 94945A213:3
- Insert:168: BV-222-106:2 ↔ 94945A213:4
- Insert:169: BV-222-119:3 ↔ 30205:2
- Insert:170: BV-222-116:3 ↔ 30205:1
- Insert:171: BV-222-119:4 ↔ 30205:4
- Insert:172: BV-222-116:4 ↔ 30205:3
- Insert:173: BV-222-116:2 ↔ 30205:6
- Insert:174: BV-222-116:1 ↔ 30205:8
- Insert:175: BV-222-119:1 ↔ 30205:7
- Insert:176: BV-222-119:2 ↔ 30205:5
- Insert:185: BV-222-116:2 ↔ 1199N323:1
- Insert:186: BV-222-119:2 ↔ 1199N323:2
- Insert:187: BV-222-119:4 ↔ 1199N323:3
- Insert:188: BV-222-116:4 ↔ 1199N323:4
- Insert:189: BV-222-116:1 ↔ 1199N323:5
- Insert:190: BV-222-119:1 ↔ 1199N323:6
- Insert:191: BV-222-119:3 ↔ 1199N323:7
- Insert:192: BV-222-116:3 ↔ 1199N323:8
- Insert:193: 30205:5 ↔ 0222-113-2:2
- Insert:194: 97260A109:2 ↔ 0222-113-2:2
- Insert:195: 30205:7 ↔ 0222-113-2:4
- Insert:196: 97260A109:1 ↔ 0222-113-2:4
- Insert:197: 30205:2 ↔ 0222-113-2:3
- Insert:198: 97260A109:4 ↔ 0222-113-2:3
- Insert:199: 30205:4 ↔ 0222-113-2:1
- Insert:200: 97260A109:3 ↔ 0222-113-2:1
- Flush:8: BV-ASM-222-103:1
- Flush:9: BV-ASM-222-103:1
- Flush:10: BV-ASM-222-103:1
- Insert:201: BV-ASM-222-103:1 ↔ BV-222-109:1
- Insert:202: BV-ASM-222-103:1 ↔ BV-222-109:1
- Insert:203: BV-ASM-222-103:2 ↔ BV-222-109:2
- Insert:204: BV-ASM-222-103:2 ↔ BV-222-109:2
- Insert:205: BV-ASM-222-103:2 ↔ Hex Flange Screw - Inch (IFI) 3/8-16 UNC x 0.625:32
- Insert:206: BV-ASM-222-103:2 ↔ Hex Flange Screw - Inch (IFI) 3/8-16 UNC x 0.625:33
- Insert:207: BV-ASM-222-103:3 ↔ BV-222-109:4
- Insert:208: BV-ASM-222-103:3 ↔ BV-222-109:4
- Insert:209: BV-ASM-222-103:3 ↔ Hex Flange Screw - Inch (IFI) 3/8-16 UNC x 0.625:36
- Insert:210: BV-ASM-222-103:3 ↔ Hex Flange Screw - Inch (IFI) 3/8-16 UNC x 0.625:37
- Insert:211: BV-ASM-222-103:4 ↔ BV-222-109:3
- Insert:212: BV-ASM-222-103:4 ↔ BV-222-109:3
- Insert:213: BV-ASM-222-103:4 ↔ Hex Flange Screw - Inch (IFI) 3/8-16 UNC x 0.625:35
- Insert:214: BV-ASM-222-103:4 ↔ Hex Flange Screw - Inch (IFI) 3/8-16 UNC x 0.625:34
- Flush:11: BV-ASM-222-104:1
- Flush:12: BV-ASM-222-104:1
- Flush:13: BV-ASM-222-104:1
- Insert:215: BV-ASM-222-102:1 ↔ 30205:1
- Mate:101: BV-ASM-222-102:4 ↔ 251105 Motor_Drive:2
- Insert:216: BV-ASM-222-102:4 ↔ 30205:6
- Mate:102: BV-ASM-222-102:2 ↔ 251105 Motor_Drive:1
- Insert:217: BV-ASM-222-102:2 ↔ 30205:8
- Mate:103: BV-ASM-222-102:3 ↔ 251105 Motor_Drive:3
- Insert:218: BV-ASM-222-102:3 ↔ 30205:3
- Insert:219: BV-ASM-222-103:2 ↔ BV-222-109:2
- Insert:220: BV-ASM-222-103:2 ↔ BV-222-109:2
- Insert:221: BV-ASM-222-103:3 ↔ BV-222-109:4
- Insert:222: BV-ASM-222-103:3 ↔ BV-222-109:4
- Insert:223: BV-ASM-222-103:4 ↔ BV-222-109:3
- Insert:224: BV-ASM-222-103:4 ↔ BV-222-109:3
- Mate:105: BV-ASM-222-105:1 ↔ 0222-110:2
## Named parameters: Boltoffset = 4.7752 mm, d214_d160 = 0 mm, d215_d161 = 0 mm, d216_d164 = 0 mm, d217_d165 = 0 mm, d220_d172 = 0 mm, d221_d173 = 0 mm, d222_d176 = 0 mm, d223_d177 = 0 mm
